# Autodesk Inventor assembly: RightHandSimpleFinger
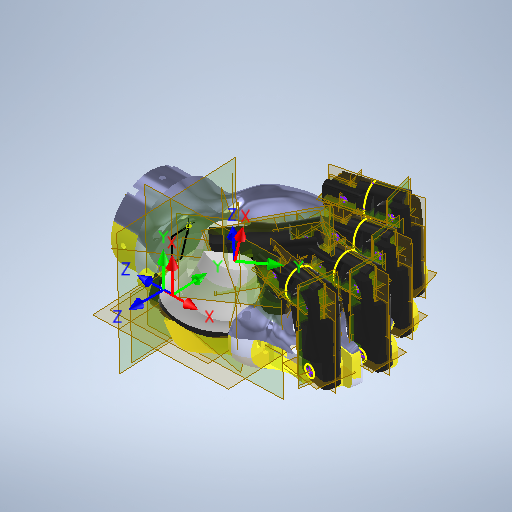
[picture p0: Inventor's stored thumbnail of the model, 512x512]
Saved by Autodesk Inventor 2025.1 (Build 291241000, 241)
## iProperties
Created: 2025-05-11
Part Number: RightHandSimpleFinger
Document SubType Name: Assembly
Designer: Alexander
Author: Alexander
## Documents named in this file (9)
- D:\Repositorios_Politecnica\Handi-EPN\CAD\Sim Models\RightHandSimpleFinger.iam
- D:\Repositorios_Politecnica\Handi-EPN\CAD\Sim Models\GenericProximalPhalanx.iam
- D:\Repositorios_Politecnica\Handi-EPN\CAD\Sim Models\GenericMiddlePhalanx.iam
- D:\Repositorios_Politecnica\Handi-EPN\CAD\Sim Models\GenericDistalPhalanx.iam
- D:\Repositorios_Politecnica\Handi-EPN\CAD\Right Hand\Dorsal Palm R Motores nuevo.ipt
- D:\Repositorios_Politecnica\Handi-EPN\CAD\Sim Models\ThumbProximalPhalanx.iam
- D:\Repositorios_Politecnica\Handi-EPN\CAD\Sim Models\ThumbMiddlePhalanx.iam
- D:\Repositorios_Politecnica\Handi-EPN\CAD\Sim Models\ThumbDistalPhalanx.iam
- D:\Repositorios_Politecnica\Handi-EPN\CAD\Right Hand\Ventral Palm R Motores Nuevo.ipt
## Components (17 placed, 8 different names)
1. GenericProximalPhalanx:1 [sub-assembly] — Rotational:1, Rotational:2
2. GenericMiddlePhalanx:1 [sub-assembly] — Rotational:2, Rotational:3
3. GenericDistalPhalanx:1 [sub-assembly] — Rotational:3
4. Dorsal Palm R Motores nuevo:6 — Rotational:1, Rotational:6, Rotational:9, Rotational:12, Mate:1, Flush:1, Flush:2, Rotational:13, Mate:2, Flush:3, Flush:4
5. GenericProximalPhalanx:2 [sub-assembly] — Rotational:6
6. GenericMiddlePhalanx:2 [sub-assembly]
7. GenericDistalPhalanx:2 [sub-assembly]
8. GenericProximalPhalanx:3 [sub-assembly] — Rotational:9
9. GenericMiddlePhalanx:3 [sub-assembly]
10. GenericDistalPhalanx:3 [sub-assembly]
11. GenericProximalPhalanx:4 [sub-assembly] — Rotational:12
12. GenericMiddlePhalanx:4 [sub-assembly]
13. GenericDistalPhalanx:4 [sub-assembly]
14. ThumbProximalPhalanx:5 [sub-assembly] — Rotational:14, Rotational:13
15. ThumbMiddlePhalanx:5 [sub-assembly] — Rotational:14, Rotational:15
16. ThumbDistalPhalanx:5 [sub-assembly] — Rotational:15
17. Ventral Palm R Motores Nuevo:1 — Mate:2, Flush:3, Flush:4
## Relationships (21: RevoluteJoint 15, Flush 4, Mate 2)
- Rotational:1 [RevoluteJoint]: GenericProximalPhalanx:1 ↔ Dorsal Palm R Motores nuevo:6
- Rotational:2 [RevoluteJoint]: GenericProximalPhalanx:1 ↔ GenericMiddlePhalanx:1
- Rotational:3 [RevoluteJoint]: GenericMiddlePhalanx:1 ↔ GenericDistalPhalanx:1
- [RevoluteJoint]: GenericProximalPhalanx:2 ↔ GenericMiddlePhalanx:2
- [RevoluteJoint]: GenericMiddlePhalanx:2 ↔ GenericDistalPhalanx:2
- Rotational:6 [RevoluteJoint]: Dorsal Palm R Motores nuevo:6 ↔ GenericProximalPhalanx:2
- [RevoluteJoint]: GenericProximalPhalanx:3 ↔ GenericMiddlePhalanx:3
- [RevoluteJoint]: GenericMiddlePhalanx:3 ↔ GenericDistalPhalanx:3
- Rotational:9 [RevoluteJoint]: Dorsal Palm R Motores nuevo:6 ↔ GenericProximalPhalanx:3
- [RevoluteJoint]: GenericProximalPhalanx:4 ↔ GenericMiddlePhalanx:4
- [RevoluteJoint]: GenericMiddlePhalanx:4 ↔ GenericDistalPhalanx:4
- Rotational:12 [RevoluteJoint]: Dorsal Palm R Motores nuevo:6 ↔ GenericProximalPhalanx:4
- Mate:1: Dorsal Palm R Motores nuevo:6
- Flush:1: Dorsal Palm R Motores nuevo:6
- Flush:2: Dorsal Palm R Motores nuevo:6
- Rotational:14 [RevoluteJoint] (-1.25 mm): ThumbProximalPhalanx:5 ↔ ThumbMiddlePhalanx:5
- Rotational:15 [RevoluteJoint] (-1.25 mm): ThumbMiddlePhalanx:5 ↔ ThumbDistalPhalanx:5
- Rotational:13 [RevoluteJoint]: Dorsal Palm R Motores nuevo:6 ↔ ThumbProximalPhalanx:5
- Mate:2: Dorsal Palm R Motores nuevo:6 ↔ Ventral Palm R Motores Nuevo:1
- Flush:3: Dorsal Palm R Motores nuevo:6 ↔ Ventral Palm R Motores Nuevo:1
- Flush:4: Dorsal Palm R Motores nuevo:6 ↔ Ventral Palm R Motores Nuevo:1
## Named parameters: d6_d2 = 0 mm, d7_d3 = -44 deg, d8_d4 = 0 mm, d9_d5 = 289 deg, d12_d6_d2 = 0 mm, d13_d7_d3 = -39 deg, d14_d8_d4 = 0 mm, d15_d9_d5 = 269.220001 deg, d18_d6_d2 = 0 mm, d19_d7_d3 = -39 deg, d20_d8_d4 = 0 mm, d21_d9_d5 = -71 deg
